# Autodesk Inventor assembly: PZT Assembly
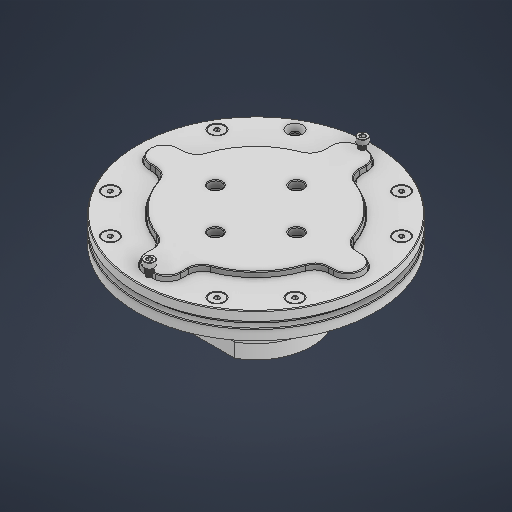
[picture p0: Inventor's stored thumbnail of the model, 512x512]
Saved by Autodesk Inventor 2025 (Build 290162000, 162)
## iProperties
Created: 2024-07-01
Part Number: PZT Assembly
Document SubType Name: Assembly
Designer: mayhe
Author: mayhe
## Documents named in this file (13)
- C:\Users\mayhe\OneDrive\Documents\GitHub\In-situ-monitoring-of-powder-bed-fusion-additive-manufacturing\system_development\Orichalcum\v0.2\Hardware_design\pzt-parts\PZT Assembly.iam
- C:\Users\mayhe\OneDrive\Documents\GitHub\In-situ-monitoring-of-powder-bed-fusion-additive-manufacturing\system_development\Orichalcum\v0.2\Hardware_design\pzt-parts\Modified Substrate Plate Bottom.ipt
- C:\Users\mayhe\OneDrive\Documents\GitHub\In-situ-monitoring-of-powder-bed-fusion-additive-manufacturing\system_development\Orichalcum\v0.2\Hardware_design\pzt-parts\Build Plateform.ipt
- C:\Users\mayhe\OneDrive\Documents\GitHub\In-situ-monitoring-of-powder-bed-fusion-additive-manufacturing\system_development\Orichalcum\v0.2\Hardware_design\pzt-parts\Clamp Ring.ipt
- C:\Users\mayhe\OneDrive\Documents\GitHub\In-situ-monitoring-of-powder-bed-fusion-additive-manufacturing\system_development\Orichalcum\v0.2\Hardware_design\pzt-parts\91292A229_18-8 Stainless Steel Socket Head Sc.ipt
- C:\Users\mayhe\OneDrive\Documents\GitHub\In-situ-monitoring-of-powder-bed-fusion-additive-manufacturing\system_development\Orichalcum\v0.2\Hardware_design\pzt-parts\91294A208_Black-Oxide Alloy Steel Hex Drive F.ipt
- C:\Users\mayhe\OneDrive\Documents\GitHub\In-situ-monitoring-of-powder-bed-fusion-additive-manufacturing\system_development\Orichalcum\v0.2\Hardware_design\pzt-parts\91290.ipt
- C:\Users\mayhe\OneDrive\Documents\GitHub\In-situ-monitoring-of-powder-bed-fusion-additive-manufacturing\system_development\Orichalcum\v0.2\Hardware_design\pzt-parts\90133A240_Oil-Resistant Neoprene Rubber Seali.ipt
- C:\Users\mayhe\OneDrive\Documents\GitHub\In-situ-monitoring-of-powder-bed-fusion-additive-manufacturing\system_development\Orichalcum\v0.2\Hardware_design\pzt-parts\94709A153_Metal-Bonded Sealing Washer with Ne.ipt
- C:\Users\mayhe\OneDrive\Documents\Inventor\Content Center Files\R2025\en-US\AS 1474(1)\AS 1474 - M8(1).ipt
- C:\Users\mayhe\OneDrive\Documents\GitHub\In-situ-monitoring-of-powder-bed-fusion-additive-manufacturing\system_development\Orichalcum\v0.2\Hardware_design\pzt-parts\Adapter Plate.ipt
- C:\Users\mayhe\OneDrive\Documents\GitHub\In-situ-monitoring-of-powder-bed-fusion-additive-manufacturing\system_development\Orichalcum\v0.2\Hardware_design\pzt-parts\PZT cell.ipt
- C:\Users\mayhe\OneDrive\Documents\GitHub\In-situ-monitoring-of-powder-bed-fusion-additive-manufacturing\system_development\Orichalcum\v0.2\Hardware_design\pzt-parts\CMG024 Transducer.ipt
## Components (41 placed, 12 different names)
1. Build Plateform:1 — Mate:1, Rotational:3, Rotational:8, Rotational:27
2. Clamp Ring:1 — Mate:1, Rotational:3, Rotational:9, Rotational:10, Rotational:11, Rotational:12, Rotational:13, Rotational:14, Rotational:15, Rotational:16
3. Modified Substrate Plate Bottom:3 — Rotational:8, Rotational:17, Rotational:18, Rotational:19, Rotational:20, Rotational:21, Rotational:22, Rotational:23, Rotational:24, Rotational:25, Rotational:26
4. PZT cell:1 — Rotational:27, Rotational:28, Rotational:29
5. Adapter Plate:1 — Rotational:29
6. CMG024 Transducer:1 — Rotational:28
7. 90133A240_Oil-Resistant Neoprene Rubber Seali:1 — Rotational:22, Insert:11
8. 90133A240_Oil-Resistant Neoprene Rubber Seali:2 — Rotational:21, Insert:10
9. 90133A240_Oil-Resistant Neoprene Rubber Seali:3 — Rotational:19, Insert:9
10. 90133A240_Oil-Resistant Neoprene Rubber Seali:4 — Rotational:20, Insert:12
11. 94709A153_Metal-Bonded Sealing Washer with Ne:1 — Rotational:25, Insert:3
12. 94709A153_Metal-Bonded Sealing Washer with Ne:2 — Rotational:26, Insert:4
13. 94709A153_Metal-Bonded Sealing Washer with Ne:3 — Rotational:23, Insert:2
14. 94709A153_Metal-Bonded Sealing Washer with Ne:4 — Rotational:24, Insert:1
15. 90133A240_Oil-Resistant Neoprene Rubber Seali:5 — Insert:5
16. 90133A240_Oil-Resistant Neoprene Rubber Seali:6 — Insert:8
17. 90133A240_Oil-Resistant Neoprene Rubber Seali:7 — Insert:6
18. 90133A240_Oil-Resistant Neoprene Rubber Seali:8 — Insert:7
19. AS 1474 - Metric M8:1 — Insert:1
20. AS 1474 - Metric M8:2 — Insert:2
21. AS 1474 - Metric M8:3 — Insert:3
22. AS 1474 - Metric M8:4 — Insert:4
23. AS 1474 - Metric M8:5 — Insert:5
24. AS 1474 - Metric M8:6 — Insert:6
25. AS 1474 - Metric M8:7 — Insert:7
26. AS 1474 - Metric M8:8 — Insert:8
27. AS 1474 - Metric M8:9 — Insert:9
28. AS 1474 - Metric M8:10 — Insert:10
29. AS 1474 - Metric M8:11 — Insert:11
30. AS 1474 - Metric M8:12 — Insert:12
31. 91292A229_18-8 Stainless Steel Socket Head Sc:1
32. 91294A208_Black-Oxide Alloy Steel Hex Drive F:1 — Rotational:9
33. 91294A208_Black-Oxide Alloy Steel Hex Drive F:2 — Rotational:10
34. 91294A208_Black-Oxide Alloy Steel Hex Drive F:3 — Rotational:11
35. 91294A208_Black-Oxide Alloy Steel Hex Drive F:4 — Rotational:12
36. 91294A208_Black-Oxide Alloy Steel Hex Drive F:5 — Rotational:15
37. 91294A208_Black-Oxide Alloy Steel Hex Drive F:6 — Rotational:16
38. 91294A208_Black-Oxide Alloy Steel Hex Drive F:7 — Rotational:13
39. 91294A208_Black-Oxide Alloy Steel Hex Drive F:8 — Rotational:14
40. 91290:1 — Rotational:17
41. 91290:2 — Rotational:18
## Relationships (36: RevoluteJoint 23, Insert 12, Mate 1)
- Mate:1: Build Plateform:1 ↔ Clamp Ring:1
- Rotational:3 [RevoluteJoint]: Build Plateform:1 ↔ Clamp Ring:1
- Rotational:8 [RevoluteJoint]: Build Plateform:1 ↔ Modified Substrate Plate Bottom:3
- Rotational:9 [RevoluteJoint]: Clamp Ring:1 ↔ 91294A208_Black-Oxide Alloy Steel Hex Drive F:1
- Rotational:10 [RevoluteJoint]: Clamp Ring:1 ↔ 91294A208_Black-Oxide Alloy Steel Hex Drive F:2
- Rotational:11 [RevoluteJoint]: Clamp Ring:1 ↔ 91294A208_Black-Oxide Alloy Steel Hex Drive F:3
- Rotational:12 [RevoluteJoint]: Clamp Ring:1 ↔ 91294A208_Black-Oxide Alloy Steel Hex Drive F:4
- Rotational:13 [RevoluteJoint]: Clamp Ring:1 ↔ 91294A208_Black-Oxide Alloy Steel Hex Drive F:7
- Rotational:14 [RevoluteJoint]: Clamp Ring:1 ↔ 91294A208_Black-Oxide Alloy Steel Hex Drive F:8
- Rotational:15 [RevoluteJoint]: Clamp Ring:1 ↔ 91294A208_Black-Oxide Alloy Steel Hex Drive F:5
- Rotational:16 [RevoluteJoint]: Clamp Ring:1 ↔ 91294A208_Black-Oxide Alloy Steel Hex Drive F:6
- Rotational:17 [RevoluteJoint]: Modified Substrate Plate Bottom:3 ↔ 91290:1
- Rotational:18 [RevoluteJoint]: Modified Substrate Plate Bottom:3 ↔ 91290:2
- Rotational:19 [RevoluteJoint]: Modified Substrate Plate Bottom:3 ↔ 90133A240_Oil-Resistant Neoprene Rubber Seali:3
- Rotational:20 [RevoluteJoint]: Modified Substrate Plate Bottom:3 ↔ 90133A240_Oil-Resistant Neoprene Rubber Seali:4
- Rotational:21 [RevoluteJoint]: Modified Substrate Plate Bottom:3 ↔ 90133A240_Oil-Resistant Neoprene Rubber Seali:2
- Rotational:22 [RevoluteJoint]: Modified Substrate Plate Bottom:3 ↔ 90133A240_Oil-Resistant Neoprene Rubber Seali:1
- Rotational:23 [RevoluteJoint]: Modified Substrate Plate Bottom:3 ↔ 94709A153_Metal-Bonded Sealing Washer with Ne:3
- Rotational:24 [RevoluteJoint]: Modified Substrate Plate Bottom:3 ↔ 94709A153_Metal-Bonded Sealing Washer with Ne:4
- Rotational:25 [RevoluteJoint]: Modified Substrate Plate Bottom:3 ↔ 94709A153_Metal-Bonded Sealing Washer with Ne:1
- Rotational:26 [RevoluteJoint]: Modified Substrate Plate Bottom:3 ↔ 94709A153_Metal-Bonded Sealing Washer with Ne:2
- Insert:1: 94709A153_Metal-Bonded Sealing Washer with Ne:4 ↔ AS 1474 - Metric M8:1
- Insert:2: 94709A153_Metal-Bonded Sealing Washer with Ne:3 ↔ AS 1474 - Metric M8:2
- Insert:3: 94709A153_Metal-Bonded Sealing Washer with Ne:1 ↔ AS 1474 - Metric M8:3
- Insert:4: 94709A153_Metal-Bonded Sealing Washer with Ne:2 ↔ AS 1474 - Metric M8:4
- Insert:5: 90133A240_Oil-Resistant Neoprene Rubber Seali:5 ↔ AS 1474 - Metric M8:5
- Insert:6: 90133A240_Oil-Resistant Neoprene Rubber Seali:7 ↔ AS 1474 - Metric M8:6
- Insert:7: 90133A240_Oil-Resistant Neoprene Rubber Seali:8 ↔ AS 1474 - Metric M8:7
- Insert:8: 90133A240_Oil-Resistant Neoprene Rubber Seali:6 ↔ AS 1474 - Metric M8:8
- Insert:9: 90133A240_Oil-Resistant Neoprene Rubber Seali:3 ↔ AS 1474 - Metric M8:9
- Insert:10: 90133A240_Oil-Resistant Neoprene Rubber Seali:2 ↔ AS 1474 - Metric M8:10
- Insert:11: 90133A240_Oil-Resistant Neoprene Rubber Seali:1 ↔ AS 1474 - Metric M8:11
- Insert:12: 90133A240_Oil-Resistant Neoprene Rubber Seali:4 ↔ AS 1474 - Metric M8:12
- Rotational:27 [RevoluteJoint]: Build Plateform:1 ↔ PZT cell:1
- Rotational:28 [RevoluteJoint]: PZT cell:1 ↔ CMG024 Transducer:1
- Rotational:29 [RevoluteJoint]: PZT cell:1 ↔ Adapter Plate:1
